# Autodesk Inventor assembly: TubeFrame
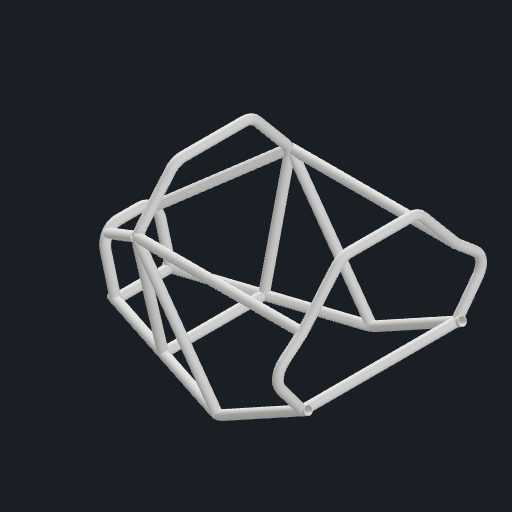
[picture p0: Inventor's stored thumbnail of the model, 512x512]
Saved by Autodesk Inventor 2025.2 (Build 292293000, 293)
## iProperties
Created: 2025-04-01
Part Number: TubeFrame
Document SubType Name: Assembly
Designer: valer
Author: valer
## Documents named in this file (2)
- C:\Users\valer\Desktop\str1ker\cad\TubeFrame.iam
- C:\Users\valer\Desktop\str1ker\cad\Chest.ipt
## Components (1 placed, 1 different names)
1. Chest:1 — Flush:1, Mate:1
## Relationships (2: Flush 1, Mate 1)
- Flush:1: Chest:1
- Mate:1: Chest:1
